# Autodesk Inventor assembly: am-2971
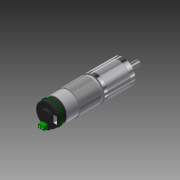
[picture p0: Inventor's stored thumbnail of the model, 180x180]
Saved by Autodesk Inventor 2016 SP1 (Build 200210100, 210)
## iProperties
Category: Motors
Company: Autodesk Inc.
Created: 2015-11-26
Part Number: am-2971
Document SubType Name: Assembly
Designer: Autodesk Inc.
Catalog Web Link: http://www.andymark.com/product-p/am-2971.htm
Vendor: AndyMark Inc.
Author: Autodesk Inc.
## Documents named in this file (3)
- D:\FIRST\FRC KOP 2016\FRC KOP 2016\Motors\MOT_GearMotEncoder_am-2971.iam
- D:\FIRST\FRC KOP 2016\FRC FIRSTChoice 2016\fc16-004_GearMotor.ipt
- D:\FIRST\FRC KOP 2016\FRC KOP 2016\Motors\Parts\Hall Effect Encoder for PG Gearboxes.ipt
## Components (2 placed, 2 different names)
1. fc16-004_GearMotor:1 — Insert:1, Angle:1
2. Hall Effect Encoder for PG Gearboxes:1 — Insert:1, Angle:1
## Relationships (2: Insert 1, Angle 1)
- Insert:1: fc16-004_GearMotor:1 ↔ Hall Effect Encoder for PG Gearboxes:1
- Angle:1 (0 deg): fc16-004_GearMotor:1 ↔ Hall Effect Encoder for PG Gearboxes:1
